# Autodesk Inventor assembly: gripperAssembly
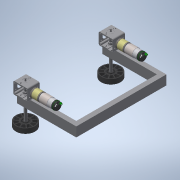
[picture p0: Inventor's stored thumbnail of the model, 180x180]
Saved by Autodesk Inventor 2022.2 (Build 262287000, 287)
## iProperties
Created: 2018-01-16
Part Number: gripperAssembly
Document SubType Name: Assembly
Designer: steele
Author: steele
## Documents named in this file (5)
- C:\git\CAD-Development\robSteele\2018-FRC\Gripper\gripperAssembly.iam
- C:\git\CAD-Development\robSteele\2018-FRC\Gripper\GripperFrame.ipt
- C:\git\CAD-Development\robSteele\2018-FRC\BevelBox\BevelGearBox.iam
- C:\git\CAD-Development\robSteele\2018-FRC\Motors\Am-2923+PG27-gearBox.iam
- C:\git\CAD-Development\robSteele\2018-FRC\Wheels\4-inch-compliantWheels.iam
## Components (7 placed, 4 different names)
1. GripperFrame:1 — Insert:2, Flush:1
2. BevelGearBox:1 [sub-assembly] — Insert:1, Insert:2, Flush:1, Insert:4
3. Am-2923+PG27-gearBox:1 [sub-assembly] — Insert:1
4. BevelGearBox:2 [sub-assembly] — Insert:3
5. Am-2923+PG27-gearBox:2 [sub-assembly] — Insert:3
6. 4-inch-compliantWheels:1 [sub-assembly] — Insert:4
7. 4-inch-compliantWheels:2 [sub-assembly]
## Relationships (5: Insert 4, Flush 1)
- Insert:1: BevelGearBox:1 ↔ Am-2923+PG27-gearBox:1
- Insert:2: GripperFrame:1 ↔ BevelGearBox:1
- Flush:1: GripperFrame:1 ↔ BevelGearBox:1
- Insert:3: BevelGearBox:2 ↔ Am-2923+PG27-gearBox:2
- Insert:4: BevelGearBox:1 ↔ 4-inch-compliantWheels:1
